# Autodesk Inventor assembly: AssemblyFile
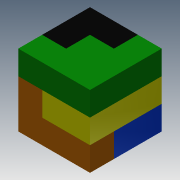
[picture p0: Inventor's stored thumbnail of the model, 180x180]
Saved by Autodesk Inventor 2015 (Build 190159000, 159)
## iProperties
Created: 2016-10-21
Part Number: AssemblyFile
Document SubType Name: Assembly
Designer: Aniket Pant
Author: Aniket Pant
## Documents named in this file (6)
- F:\Autodesk - 3D Models\IED\PuzzleCubeProject\Assemblies\AssemblyFile.iam
- F:\Autodesk - 3D Models\IED\PuzzleCubeProject\PuzzleCubeModels\GreenPuzzlePiece.ipt
- F:\Autodesk - 3D Models\IED\PuzzleCubeProject\PuzzleCubeModels\YellowPuzzlePiece.ipt
- F:\Autodesk - 3D Models\IED\PuzzleCubeProject\PuzzleCubeModels\OrangePuzzlePiece.ipt
- F:\Autodesk - 3D Models\IED\PuzzleCubeProject\PuzzleCubeModels\BluePuzzlePiece.ipt
- F:\Autodesk - 3D Models\IED\PuzzleCubeProject\PuzzleCubeModels\BlackPuzzlePiece.ipt
## Components (5 placed, 5 different names)
1. GreenPuzzlePiece — Mate:1, Flush:1, Flush:2, Flush:3, Flush:4, Mate:2, Flush:20
2. YellowPuzzlePiece:1 — Mate:1, Flush:1, Flush:2, Flush:3, Flush:4, Flush:5, Flush:6, Flush:7, Flush:9, Flush:10, Flush:11, Flush:12, Flush:16, Flush:17, Flush:21
3. OrangePuzzlePiece:1 — Mate:2, Flush:5, Flush:6, Flush:7, Mate:3, Flush:8, Flush:13, Flush:14, Flush:15
4. BluePuzzlePiece:1 — Mate:3, Flush:8, Flush:9, Flush:10, Flush:11, Flush:12, Flush:13, Flush:14, Flush:15, Flush:16, Flush:17, Mate:4, Flush:18, Flush:19
5. BlackPuzzlePiece:1 — Mate:4, Flush:18, Flush:19, Flush:20, Flush:21
## Relationships (25: Flush 21, Mate 4)
- Mate:1: GreenPuzzlePiece ↔ YellowPuzzlePiece:1
- Flush:1: GreenPuzzlePiece ↔ YellowPuzzlePiece:1
- Flush:2: GreenPuzzlePiece ↔ YellowPuzzlePiece:1
- Flush:3: GreenPuzzlePiece ↔ YellowPuzzlePiece:1
- Flush:4: GreenPuzzlePiece ↔ YellowPuzzlePiece:1
- Mate:2: GreenPuzzlePiece ↔ OrangePuzzlePiece:1
- Flush:5: YellowPuzzlePiece:1 ↔ OrangePuzzlePiece:1
- Flush:6: YellowPuzzlePiece:1 ↔ OrangePuzzlePiece:1
- Flush:7: YellowPuzzlePiece:1 ↔ OrangePuzzlePiece:1
- Mate:3: OrangePuzzlePiece:1 ↔ BluePuzzlePiece:1
- Flush:8: OrangePuzzlePiece:1 ↔ BluePuzzlePiece:1
- Flush:9: YellowPuzzlePiece:1 ↔ BluePuzzlePiece:1
- Flush:10: YellowPuzzlePiece:1 ↔ BluePuzzlePiece:1
- Flush:11: YellowPuzzlePiece:1 ↔ BluePuzzlePiece:1
- Flush:12: YellowPuzzlePiece:1 ↔ BluePuzzlePiece:1
- Flush:13: OrangePuzzlePiece:1 ↔ BluePuzzlePiece:1
- Flush:14: OrangePuzzlePiece:1 ↔ BluePuzzlePiece:1
- Flush:15: OrangePuzzlePiece:1 ↔ BluePuzzlePiece:1
- Flush:16: YellowPuzzlePiece:1 ↔ BluePuzzlePiece:1
- Flush:17: YellowPuzzlePiece:1 ↔ BluePuzzlePiece:1
- Mate:4: BluePuzzlePiece:1 ↔ BlackPuzzlePiece:1
- Flush:18: BluePuzzlePiece:1 ↔ BlackPuzzlePiece:1
- Flush:19: BluePuzzlePiece:1 ↔ BlackPuzzlePiece:1
- Flush:20: GreenPuzzlePiece ↔ BlackPuzzlePiece:1
- Flush:21: YellowPuzzlePiece:1 ↔ BlackPuzzlePiece:1
